# Autodesk Inventor assembly: ASY PNS 1220 frame right floor
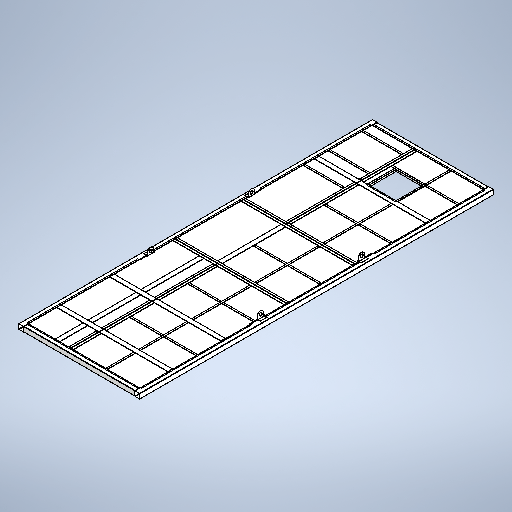
[picture p0: Inventor's stored thumbnail of the model, 512x512]
Saved by Autodesk Inventor 2025.3 (Build 293356030, 356C)
## iProperties
Created: 2025-03-15
Part Number: ASY PNS 1220 frame right floor
Document SubType Name: Assembly
Designer: admin
Mass: 658050 g
Surface Area: 604170 cm^2
Volume: 83312 cm^3
Density: 7.89861 g/cm^3
_SolveAssemblyDoc: Frame Generator Solve Assembly
_Version: 25.0.0
Author: admin
## Documents named in this file (10)
- C:\Users\admin\Yandex.Disk\home pc\Inventor\PNS2-Panaevsk\ASY PNS 1220 frame right floor.iam
- C:\Users\admin\Yandex.Disk\home pc\Inventor\PNS2-Panaevsk\PNS-0210 frame right floor Sketch.ipt
- C:\Users\admin\Yandex.Disk\home pc\Inventor\PNS2-Panaevsk\ASY PNS-0210 frame right floor\Frame\Frame 1742033625963.iam
- C:\Users\admin\Yandex.Disk\home pc\Inventor\PNS2-Panaevsk\PNS-0111 floor sheet 2.ipt
- C:\Users\admin\Yandex.Disk\home pc\Inventor\PNS2-Panaevsk\PNS-0810 floor ring.ipt
- C:\Users\admin\Yandex.Disk\home pc\Inventor\PNS2-Panaevsk\PNS-0812 floor ring  strengthen.ipt
- C:\Users\admin\Yandex.Disk\home pc\Inventor\PNS2-Panaevsk\PNS-0113 floor sheet 31.ipt
- C:\Users\admin\Yandex.Disk\home pc\Inventor\PNS2-Panaevsk\PNS-0114 floor sheet 41.ipt
- C:\Users\admin\Yandex.Disk\home pc\Inventor\PNS2-Panaevsk\PNS-0115 floor sheet 5.ipt
- C:\Users\admin\Yandex.Disk\home pc\Inventor\PNS2-Panaevsk\PNS-0116 floor sheet 6.ipt
## Components (15 placed, 9 different names)
1. PNS-0210 frame right floor Sketch:1 — Mate:24
2. Frame 1742033625963:1 [sub-assembly] — Mate:1, Flush:1, Flush:2, Mate:17, Mate:18, Mate:19, Flush:6, Flush:7, Mate:20, Flush:8, Flush:9, Mate:21, Flush:10, Flush:11, Mate:22, Flush:12
3. PNS-0111 floor sheet 2:3 — Mate:1, Flush:1, Flush:2
4. PNS-0812 floor ring  strengthen:2
5. PNS-0810 floor ring:2
6. PNS-0810 floor ring:3
7. PNS-0812 floor ring  strengthen:3 — Mate:17
8. PNS-0812 floor ring  strengthen:4 — Mate:18
9. PNS-0810 floor ring:4
10. PNS-0812 floor ring  strengthen:1
11. PNS-0810 floor ring:1
12. PNS-0113 floor sheet 3:1 — Mate:19, Flush:6, Flush:7
13. PNS-0114 floor sheet 41:1 — Mate:20, Flush:8, Flush:9
14. PNS-0115 floor sheet 5:1 — Mate:21, Flush:10, Flush:11, Mate:23
15. PNS-0116 floor sheet 6:1 — Mate:22, Flush:12, Mate:23
## Relationships (40: Mate 24, Flush 12, Tangent 4)
- Mate:1: Frame 1742033625963:1 ↔ PNS-0111 floor sheet 2:3
- Flush:1 (70 mm): Frame 1742033625963:1 ↔ PNS-0111 floor sheet 2:3
- Flush:2 (70 mm): Frame 1742033625963:1 ↔ PNS-0111 floor sheet 2:3
- [Mate] (6 mm): Frame 1742033625963:1 ↔ PNS-0810 floor ring:1
- [Tangent] (20 mm): Frame 1742033625963:1 ↔ PNS-0810 floor ring:1
- [Mate]: Frame 1742033625963:1 ↔ PNS-0812 floor ring  strengthen:1
- [Mate]: Frame 1742033625963:1 ↔ PNS-0812 floor ring  strengthen:1
- [Flush]: PNS-0812 floor ring  strengthen:1 ↔ PNS-0810 floor ring:1
- [Mate]: PNS-0812 floor ring  strengthen:2 ↔ PNS-0810 floor ring:2
- [Mate]: PNS-0812 floor ring  strengthen:2 ↔ PNS-0810 floor ring:2
- [Mate]: Frame 1742033625963:1 ↔ PNS-0812 floor ring  strengthen:2
- [Mate]: Frame 1742033625963:1 ↔ PNS-0812 floor ring  strengthen:2
- [Tangent] (20 mm): PNS-0812 floor ring  strengthen:2 ↔ PNS-0810 floor ring:2
- [Mate]: PNS-0810 floor ring:3 ↔ PNS-0812 floor ring  strengthen:3
- [Mate]: PNS-0810 floor ring:3 ↔ PNS-0812 floor ring  strengthen:3
- [Tangent] (20 mm): PNS-0810 floor ring:3 ↔ PNS-0812 floor ring  strengthen:3
- [Mate]: Frame 1742033625963:1 ↔ PNS-0812 floor ring  strengthen:3
- [Mate]: Frame 1742033625963:1 ↔ PNS-0812 floor ring  strengthen:3
- [Flush]: PNS-0812 floor ring  strengthen:2 ↔ PNS-0812 floor ring  strengthen:3
- [Mate]: PNS-0812 floor ring  strengthen:4 ↔ PNS-0810 floor ring:4
- [Mate]: PNS-0812 floor ring  strengthen:4 ↔ PNS-0810 floor ring:4
- [Tangent] (20 mm): PNS-0812 floor ring  strengthen:4 ↔ PNS-0810 floor ring:4
- [Mate]: Frame 1742033625963:1 ↔ PNS-0812 floor ring  strengthen:4
- [Mate]: Frame 1742033625963:1 ↔ PNS-0812 floor ring  strengthen:4
- [Flush]: PNS-0812 floor ring  strengthen:4 ↔ PNS-0812 floor ring  strengthen:1
- Mate:17 (30 mm): Frame 1742033625963:1 ↔ PNS-0812 floor ring  strengthen:3
- Mate:18 (35 mm): Frame 1742033625963:1 ↔ PNS-0812 floor ring  strengthen:4
- Mate:19: Frame 1742033625963:1 ↔ PNS-0113 floor sheet 3:1
- Flush:6 (70 mm): Frame 1742033625963:1 ↔ PNS-0113 floor sheet 3:1
- Flush:7 (70 mm): Frame 1742033625963:1 ↔ PNS-0113 floor sheet 3:1
- Mate:20: Frame 1742033625963:1 ↔ PNS-0114 floor sheet 41:1
- Flush:8 (70 mm): Frame 1742033625963:1 ↔ PNS-0114 floor sheet 41:1
- Flush:9 (70 mm): Frame 1742033625963:1 ↔ PNS-0114 floor sheet 41:1
- Mate:21: Frame 1742033625963:1 ↔ PNS-0115 floor sheet 5:1
- Flush:10 (70 mm): Frame 1742033625963:1 ↔ PNS-0115 floor sheet 5:1
- Flush:11 (70 mm): Frame 1742033625963:1 ↔ PNS-0115 floor sheet 5:1
- Mate:22: Frame 1742033625963:1 ↔ PNS-0116 floor sheet 6:1
- Flush:12 (70 mm): Frame 1742033625963:1 ↔ PNS-0116 floor sheet 6:1
- Mate:23 (10 mm): PNS-0115 floor sheet 5:1 ↔ PNS-0116 floor sheet 6:1
- Mate:24: PNS-0210 frame right floor Sketch:1
## Named parameters: d68_d63_d62 = 0 mm, d69_d66 = 0 mm, d95_d68_d63_d62 = 0 mm, d96_d69_d66 = 0 mm, d97_d72 = 20 mm, d101_d95_d68_d63_d62 = 0 mm, d102_d96_d69_d66 = 0 mm, d103_d97_d72 = 20 mm
